# Autodesk Inventor assembly: WemosLightSwitch
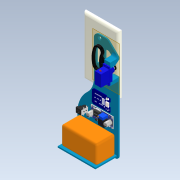
[picture p0: Inventor's stored thumbnail of the model, 180x180]
Saved by Autodesk Inventor 2020.2 (Build 242310000, 310)
## iProperties
Created: 2020-04-30
Part Number: WemosLightSwitch
Document SubType Name: Assembly
Designer: Haashim Rehan
Author: Haashim Rehan
## Documents named in this file (9)
- C:\Users\Dell\Desktop\WemosLightSwitch\WemosLightSwitch.iam
- C:\Users\Dell\Desktop\WemosLightSwitch\Light Switch Cover.ipt
- C:\Users\Dell\Desktop\WemosLightSwitch\WEMOS D1 mini.ipt
- C:\Users\Dell\Desktop\WemosLightSwitch\ble_switch_mount.ipt
- C:\Users\Dell\Desktop\WemosLightSwitch\Servo\microservoAssembly.iam
- C:\Users\Dell\Desktop\WemosLightSwitch\BatteryV1.ipt
- C:\Users\Dell\Desktop\WemosLightSwitch\LM2596 DC-DC StepDown Converter v2.iam
- C:\Users\Dell\Desktop\WemosLightSwitch\BarrelJack.ipt
- C:\Users\Dell\Desktop\WemosLightSwitch\MainBase.ipt
## Components (8 placed, 8 different names)
1. Light Switch Cover:1 — Mate:6, Mate:7, Mate:8
2. WEMOS D1 mini:2
3. MainBase:1 — Mate:4, Mate:5, Angle:1, Mate:6, Mate:7, Mate:8
4. microservoAssembly:1 [sub-assembly] — Mate:4, Mate:5, Angle:1
5. BatteryV1:1
6. LM2596 DC-DC StepDown Converter v2:1 [sub-assembly]
7. BarrelJack:1
8. ble_switch_mount:1
## Relationships (6: Mate 5, Angle 1)
- Mate:4: MainBase:1 ↔ microservoAssembly:1
- Mate:5: MainBase:1 ↔ microservoAssembly:1
- Angle:1 (0 deg): MainBase:1 ↔ microservoAssembly:1
- Mate:6: Light Switch Cover:1 ↔ MainBase:1
- Mate:7: Light Switch Cover:1 ↔ MainBase:1
- Mate:8: Light Switch Cover:1 ↔ MainBase:1
